# Autodesk Inventor assembly: Red Alliance Arm
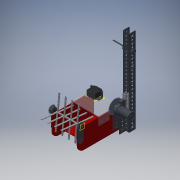
[picture p0: Inventor's stored thumbnail of the model, 180x180]
Saved by Autodesk Inventor 2016 (Build 200138000, 138)
## iProperties
Created: 2015-12-20
Part Number: Red Alliance Arm
Document SubType Name: Assembly
Designer: tbloo
Author: tbloo
## Documents named in this file (11)
- C:\Users\tbloo\Documents\GitHub\phi_robotics\3d-models\FTC_Tetrix_KOP_Block_Party\Tim Bloot Designs\JAr JaR Bot\Blue Alliance Arm.iam
- C:\Users\tbloo\Documents\GitHub\phi_robotics\3d-models\FTC_Tetrix_KOP_Block_Party\Tetrix_Kit_FTC\Autodesk Inventor Files\tetrix_c_channel-5.ipt
- C:\Users\tbloo\Documents\GitHub\phi_robotics\3d-models\FTC_Tetrix_KOP_Block_Party\Tetrix_Kit_FTC\Autodesk Inventor Files\tetrix_axle.ipt
- C:\Users\tbloo\Documents\GitHub\phi_robotics\3d-models\FTC_Tetrix_KOP_Block_Party\Tim Bloot Designs\JAr JaR Bot\Red Alliance Bucket.iam
- C:\Users\tbloo\Documents\GitHub\phi_robotics\3d-models\FTC_Tetrix_KOP_Block_Party\Tetrix_Kit_FTC\Autodesk Inventor Files\tetrix_axle_lock.iam
- C:\Users\tbloo\Documents\GitHub\phi_robotics\3d-models\FTC_Tetrix_KOP_Block_Party\Tim Bloot Designs\JAr JaR Bot\cube channel short.ipt
- C:\Users\tbloo\Documents\GitHub\phi_robotics\3d-models\FTC_Tetrix_KOP_Block_Party\Tetrix_Kit_FTC\Autodesk Inventor Files\tetrix_motor_mount-old.ipt
- C:\Users\tbloo\Documents\GitHub\phi_robotics\3d-models\FTC_Tetrix_KOP_Block_Party\Tetrix_Kit_FTC\Autodesk Inventor Files\tetrix_motor.iam
- C:\Users\tbloo\Documents\GitHub\phi_robotics\3d-models\FTC_Tetrix_KOP_Block_Party\Tetrix_Kit_FTC\Autodesk Inventor Files\tetrix_maxle_lock.iam
- C:\Users\tbloo\Documents\GitHub\phi_robotics\3d-models\FTC_Tetrix_KOP_Block_Party\Tetrix_Kit_FTC\Autodesk Inventor Files\tetrix_chain_gear-32t.ipt
- C:\Users\tbloo\Documents\GitHub\phi_robotics\3d-models\FTC_Tetrix_KOP_Block_Party\Tetrix_Kit_FTC\Autodesk Inventor Files\tetrix_c_channel-2.ipt
## Components (11 placed, 10 different names)
1. tetrix_c_channel-5:1 — Rigid:3, Rigid:4, Rigid:6, Rigid:11
2. tetrix_axle:1 — Rigid:5
3. Red Alliance Bucket:1 [sub-assembly] — Mate:1, Flush:1, Flush:2
4. tetrix_axle_lock:1 [sub-assembly] — Rigid:3, Rigid:5
5. tetrix_axle_lock:2 [sub-assembly] — Rigid:4
6. cube channel short:1 — Rigid:6, Rigid:10
7. tetrix_motor_mount-old:1 — Rigid:10, Rotational:1
8. tetrix_motor:1 [sub-assembly] — Rigid:9, Rotational:1
9. tetrix_maxle_lock:1 [sub-assembly] — Rigid:9
10. tetrix_chain_gear-32t:1
11. tetrix_c_channel-2:1 — Rigid:11, Mate:1, Flush:1, Flush:2
## Relationships (12: WeldJoint 8, Flush 2, RevoluteJoint 1, Mate 1)
- Rigid:3 [WeldJoint]: tetrix_c_channel-5:1 ↔ tetrix_axle_lock:1
- Rigid:4 [WeldJoint]: tetrix_c_channel-5:1 ↔ tetrix_axle_lock:2
- Rigid:5 [WeldJoint]: tetrix_axle:1 ↔ tetrix_axle_lock:1
- Rigid:6 [WeldJoint]: tetrix_c_channel-5:1 ↔ cube channel short:1
- [WeldJoint]: tetrix_maxle_lock:1 ↔ tetrix_chain_gear-32t:1
- Rigid:9 [WeldJoint] (-7 mm): tetrix_motor:1 ↔ tetrix_maxle_lock:1
- Rigid:10 [WeldJoint]: cube channel short:1 ↔ tetrix_motor_mount-old:1
- Rotational:1 [RevoluteJoint]: tetrix_motor_mount-old:1 ↔ tetrix_motor:1
- Rigid:11 [WeldJoint]: tetrix_c_channel-5:1 ↔ tetrix_c_channel-2:1
- Mate:1: Red Alliance Bucket:1 ↔ tetrix_c_channel-2:1
- Flush:1 (10 mm): Red Alliance Bucket:1 ↔ tetrix_c_channel-2:1
- Flush:2: Red Alliance Bucket:1 ↔ tetrix_c_channel-2:1
## Named parameters: d13_d12 = 0 mm
